# Autodesk Inventor assembly: project
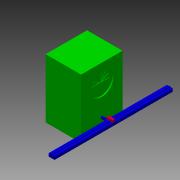
[picture p0: Inventor's stored thumbnail of the model, 180x180]
Saved by Autodesk Inventor 2015 (Build 190159000, 159)
## iProperties
Created: 2017-04-05
Part Number: project
Document SubType Name: Assembly
Designer: Mohalla
Author: Mohalla
## Documents named in this file (4)
- E:\5th\xmy work\s2\simmech\mini-project\project.iam
- E:\5th\xmy work\s2\simmech\mini-project\holder.ipt
- E:\5th\xmy work\s2\simmech\mini-project\peam.ipt
- E:\5th\xmy work\s2\simmech\mini-project\block.ipt
## Components (3 placed, 3 different names)
1. holder:1 — Mate:1, Mate:2
2. peam:1 — Mate:1, Mate:2, Mate:3, Mate:5
3. block:1 — Mate:3, Mate:5
## Relationships (4: Mate 4)
- Mate:1: holder:1 ↔ peam:1
- Mate:2: holder:1 ↔ peam:1
- Mate:3: peam:1 ↔ block:1
- Mate:5: peam:1 ↔ block:1
